# Autodesk Inventor assembly: Turret ASM
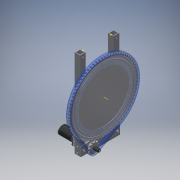
[picture p0: Inventor's stored thumbnail of the model, 180x180]
Saved by Autodesk Inventor 2017 (Build 210142000, 142)
## iProperties
Created: 2016-09-26
Part Number: Turret ASM
Document SubType Name: Assembly
Designer: Hanson
Author: Hanson
## Documents named in this file (13)
- E:\CAD\Turret\Turret ASM.iam
- E:\CAD\Turret\User Library-LazySusan 12inch.ipt
- E:\CAD\Turret\Large crossbeam.ipt
- E:\CAD\Turret\90480A195_LOW-STRENGTH STEEL HEX NUT.ipt
- E:\CAD\Turret\VEXpro-VersaPlanetary-2stage-with-BAG.iam
- E:\CAD\Turret\92196A277_18-8 STAINLESS STEEL SOCKET HEAD CAP SCREW.ipt
- E:\CAD\Turret\BAG motor top plate.ipt
- E:\CAD\Turret\92196A545_18-8 STAINLESS STEEL SOCKET HEAD CAP SCREW.ipt
- E:\CAD\Turret\plate mount nut.ipt
- E:\CAD\Turret\Main base bolt.ipt
- E:\CAD\Turret\lazy susan bushing.ipt
- E:\CAD\Turret\2737T134_FINISHED-BORE SPROCKET FOR ANSI ROLLER CHAIN.ipt
- E:\CAD\Turret\Turret ASM\Design Accelerator\Chain Drive1.iam
## Components (25 placed, 12 different names)
1. User Library-LazySusan 12inch:1 — Mate:1, Insert:25, Insert:26, Insert:27, Insert:28
2. Large crossbeam:1 — Insert:16, Insert:17, Insert:18, Insert:21, Insert:22
3. Large crossbeam:2 — Insert:13, Insert:14, Insert:15, Insert:19, Insert:20, Insert:23, Insert:24
4. VEXpro-VersaPlanetary-2stage-with-BAG:1 [sub-assembly]
5. 92196A277_18-8 STAINLESS STEEL SOCKET HEAD CAP SCREW:1 — Insert:13
6. 92196A277_18-8 STAINLESS STEEL SOCKET HEAD CAP SCREW:2 — Insert:14
7. BAG motor top plate:1 — Insert:11, Insert:12, Mate:2
8. 92196A545_18-8 STAINLESS STEEL SOCKET HEAD CAP SCREW:1 — Insert:11
9. 92196A545_18-8 STAINLESS STEEL SOCKET HEAD CAP SCREW:2 — Insert:12
10. plate mount nut:1 — Insert:15
11. plate mount nut:2 — Insert:16
12. Main base bolt:1 — Insert:17
13. Main base bolt:2 — Insert:18
14. Main base bolt:3 — Insert:19
15. Main base bolt:4 — Insert:20
16. lazy susan bushing:1 — Insert:21
17. lazy susan bushing:2 — Insert:22
18. lazy susan bushing:3 — Insert:23
19. lazy susan bushing:4 — Insert:24, Mate:1
20. 90480A195_LOW-STRENGTH STEEL HEX NUT:1 — Insert:28
21. 90480A195_LOW-STRENGTH STEEL HEX NUT:2 — Insert:27
22. 90480A195_LOW-STRENGTH STEEL HEX NUT:3 — Insert:25
23. 90480A195_LOW-STRENGTH STEEL HEX NUT:4 — Insert:26
24. 2737T134_FINISHED-BORE SPROCKET FOR ANSI ROLLER CHAIN:1 — Mate:2
25. Chain Drive:1 [sub-assembly]
## Relationships (20: Insert 18, Mate 2)
- Insert:11: BAG motor top plate:1 ↔ 92196A545_18-8 STAINLESS STEEL SOCKET HEAD CAP SCREW:1
- Insert:12: BAG motor top plate:1 ↔ 92196A545_18-8 STAINLESS STEEL SOCKET HEAD CAP SCREW:2
- Insert:13: Large crossbeam:2 ↔ 92196A277_18-8 STAINLESS STEEL SOCKET HEAD CAP SCREW:1
- Insert:14: Large crossbeam:2 ↔ 92196A277_18-8 STAINLESS STEEL SOCKET HEAD CAP SCREW:2
- Insert:15: Large crossbeam:2 ↔ plate mount nut:1
- Insert:16: Large crossbeam:1 ↔ plate mount nut:2
- Insert:17: Large crossbeam:1 ↔ Main base bolt:1
- Insert:18: Large crossbeam:1 ↔ Main base bolt:2
- Insert:19: Large crossbeam:2 ↔ Main base bolt:3
- Insert:20: Large crossbeam:2 ↔ Main base bolt:4
- Insert:21: Large crossbeam:1 ↔ lazy susan bushing:1
- Insert:22: Large crossbeam:1 ↔ lazy susan bushing:2
- Insert:23: Large crossbeam:2 ↔ lazy susan bushing:3
- Insert:24: Large crossbeam:2 ↔ lazy susan bushing:4
- Mate:1: User Library-LazySusan 12inch:1 ↔ lazy susan bushing:4
- Insert:25: User Library-LazySusan 12inch:1 ↔ 90480A195_LOW-STRENGTH STEEL HEX NUT:3
- Insert:26: User Library-LazySusan 12inch:1 ↔ 90480A195_LOW-STRENGTH STEEL HEX NUT:4
- Insert:27: User Library-LazySusan 12inch:1 ↔ 90480A195_LOW-STRENGTH STEEL HEX NUT:2
- Insert:28: User Library-LazySusan 12inch:1 ↔ 90480A195_LOW-STRENGTH STEEL HEX NUT:1
- Mate:2: BAG motor top plate:1 ↔ 2737T134_FINISHED-BORE SPROCKET FOR ANSI ROLLER CHAIN:1
